# Autodesk Inventor assembly: Ensamblaje
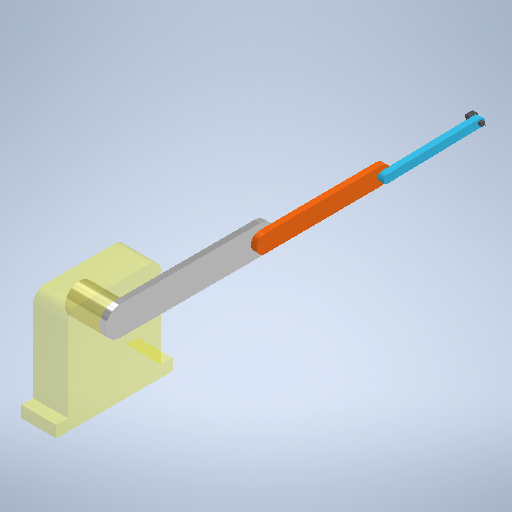
[picture p0: Inventor's stored thumbnail of the model, 512x512]
Saved by Autodesk Inventor 2025 (Build 290162000, 162)
## iProperties
Created: 2023-05-06
Part Number: Ensamblaje
Document SubType Name: Assembly
Designer: Miguel Ángel
Author: Miguel Ángel
## Documents named in this file (6)
- C:\Users\Usuario\Desktop\UA\UA\Cuatri2\Mecanismos y Modelado\Prácticas\P3\entrega\Ensamblaje.iam
- C:\Users\Usuario\Desktop\UA\UA\Cuatri2\Mecanismos y Modelado\Prácticas\P3\entrega\Base.ipt
- C:\Users\Usuario\Desktop\UA\UA\Cuatri2\Mecanismos y Modelado\Prácticas\P3\entrega\L1.ipt
- C:\Users\Usuario\Desktop\UA\UA\Cuatri2\Mecanismos y Modelado\Prácticas\P3\entrega\L2.ipt
- C:\Users\Usuario\Desktop\UA\UA\Cuatri2\Mecanismos y Modelado\Prácticas\P3\entrega\L3.ipt
- C:\Users\Usuario\Desktop\UA\UA\Cuatri2\Mecanismos y Modelado\Prácticas\P3\entrega\Herramienta.ipt
## Components (5 placed, 5 different names)
1. Base:1 — Insertar:1
2. L1:1 — Insertar:1, Insertar:2
3. L2:1 — Insertar:2, Insertar:3
4. L3:1 — Insertar:3, Rígido:1
5. Herramienta:1 — Rígido:1
## Relationships (4: Insert 3, WeldJoint 1)
- Insertar:1: Base:1 ↔ L1:1
- Insertar:2: L1:1 ↔ L2:1
- Insertar:3: L2:1 ↔ L3:1
- Rígido:1 [WeldJoint]: L3:1 ↔ Herramienta:1
